# Autodesk Inventor assembly: 0329
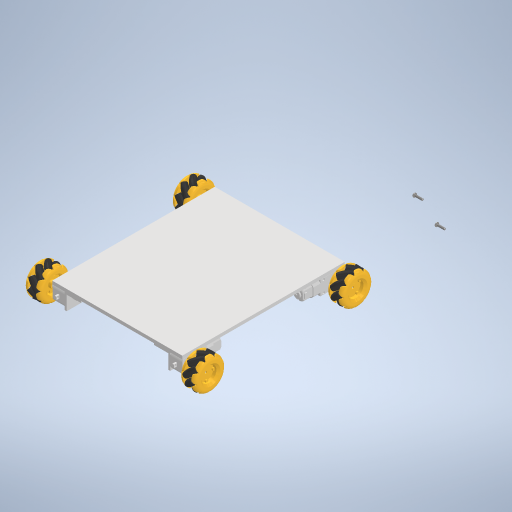
[picture p0: Inventor's stored thumbnail of the model, 512x512]
Saved by Autodesk Inventor 2023.2 (Build 272271030, 271C)
## iProperties
Created: 2023-03-29
Part Number: 0329
Document SubType Name: Assembly
Designer: kao91
Author: kao91
## Documents named in this file (9)
- C:\Users\kao91\Desktop\Mecharonic_practice\0329.iam
- C:\Users\kao91\Desktop\Mecharonic_practice\dc-motor-gearbox-tt-motor-1.snapshot.2\DC Motor Gearbox\DC Motor Gearbox.ipt
- C:\Users\kao91\Desktop\Mecharonic_practice\platform.ipt
- C:\Users\kao91\Desktop\Mecharonic_practice\connector.ipt
- C:\Users\kao91\OneDrive\文件\Inventor\Content Center Files\R2023\en-US\AS 1427(05)\AS 1427 - M3 x 12(5) II.ipt
- C:\Users\kao91\Desktop\Mecharonic_practice\df-robot-48mm-mecanum-wheel-left-side-1.snapshot.2\Mecanum Left v5\Mecanum Left v5.ipt
- C:\Users\kao91\Desktop\Mecharonic_practice\df-robot-48mm-mecanum-wheel-left-side-1.snapshot.2\Mecanum Left v5\Mecanum Ra.ipt
- C:\Users\kao91\Desktop\Mecharonic_practice\df-robot-48mm-mecanum-wheel-left-side-1.snapshot.2\Mecanum Left v5\Mecanum Rb.ipt
- C:\Users\kao91\Desktop\Mecharonic_practice\motor_to_mecanum_connector.ipt
## Components (19 placed, 8 different names)
1. platform:1 — Mate:1, Mate:2, Mate:3, Mate:4, Flush:2, Flush:3, Mate:5, Mate:7, Mate:9, Mate:11, Flush:4, Flush:5, Flush:6, Flush:7, Flush:8
2. connector:1 — Flush:3, Mate:5, Mate:6
3. connector:2 — Mate:7, Mate:8
4. connector:3 — Mate:9, Flush:5, Mate:13
5. connector:4 — Mate:11, Flush:4, Mate:14
6. AS 1427 H - Metric M3 x 12:1
7. AS 1427 H - Metric M3 x 12:2
8. DC Motor Gearbox:3 — Mate:3, Mate:13, Flush:8, Cylindrical:4, Mate:16, Flush:9
9. motor_to_mecanum_connector:4 — Cylindrical:4, Mate:16, Cylindrical:7, Mate:20
10. Mecanum Left v5:2 — Cylindrical:7, Mate:20
11. DC Motor Gearbox:1 — Mate:1, Mate:8, Flush:6, Cylindrical:2, Mate:18, Flush:10
12. motor_to_mecanum_connector:1 — Cylindrical:2, Mate:18, Cylindrical:8, Mate:22
13. Mecanum Left v5:1 — Cylindrical:8, Mate:22
14. DC Motor Gearbox:4 — Mate:4, Mate:14, Flush:7, Cylindrical:3, Mate:17, Flush:9
15. motor_to_mecanum_connector:3 — Cylindrical:3, Mate:17, Cylindrical:5, Mate:19
16. Mecanum Ra:1 — Cylindrical:5, Mate:19
17. DC Motor Gearbox:2 — Mate:2, Flush:2, Mate:6, Cylindrical:1, Mate:15, Flush:10
18. motor_to_mecanum_connector:2 — Cylindrical:1, Mate:15, Cylindrical:6, Mate:21
19. Mecanum Rb:1 — Cylindrical:6, Mate:21
## Relationships (37: Mate 20, Flush 9, CylindricalJoint 8)
- Mate:1: platform:1 ↔ DC Motor Gearbox:1
- Mate:2: platform:1 ↔ DC Motor Gearbox:2
- Mate:3: platform:1 ↔ DC Motor Gearbox:3
- Mate:4: platform:1 ↔ DC Motor Gearbox:4
- Flush:2: platform:1 ↔ DC Motor Gearbox:2
- Flush:3: platform:1 ↔ connector:1
- Mate:5: platform:1 ↔ connector:1
- Mate:6: connector:1 ↔ DC Motor Gearbox:2
- Mate:7: platform:1 ↔ connector:2
- Mate:8: connector:2 ↔ DC Motor Gearbox:1
- Mate:9: platform:1 ↔ connector:3
- Mate:11: platform:1 ↔ connector:4
- Flush:4: platform:1 ↔ connector:4
- Flush:5: platform:1 ↔ connector:3
- Flush:6: platform:1 ↔ DC Motor Gearbox:1
- Mate:13: connector:3 ↔ DC Motor Gearbox:3
- Mate:14: connector:4 ↔ DC Motor Gearbox:4
- Flush:7: platform:1 ↔ DC Motor Gearbox:4
- Cylindrical:1: DC Motor Gearbox:2 ↔ motor_to_mecanum_connector:2
- Mate:15: DC Motor Gearbox:2 ↔ motor_to_mecanum_connector:2
- Cylindrical:2: DC Motor Gearbox:1 ↔ motor_to_mecanum_connector:1
- Cylindrical:3: DC Motor Gearbox:4 ↔ motor_to_mecanum_connector:3
- Flush:8: platform:1 ↔ DC Motor Gearbox:3
- Cylindrical:4: DC Motor Gearbox:3 ↔ motor_to_mecanum_connector:4
- Mate:16: DC Motor Gearbox:3 ↔ motor_to_mecanum_connector:4
- Mate:17: DC Motor Gearbox:4 ↔ motor_to_mecanum_connector:3
- Mate:18: DC Motor Gearbox:1 ↔ motor_to_mecanum_connector:1
- Cylindrical:5: motor_to_mecanum_connector:3 ↔ Mecanum Ra:1
- Mate:19: motor_to_mecanum_connector:3 ↔ Mecanum Ra:1
- Cylindrical:6: motor_to_mecanum_connector:2 ↔ Mecanum Rb:1
- Cylindrical:7: motor_to_mecanum_connector:4 ↔ Mecanum Left v5:2
- Cylindrical:8: motor_to_mecanum_connector:1 ↔ Mecanum Left v5:1
- Mate:20: motor_to_mecanum_connector:4 ↔ Mecanum Left v5:2
- Mate:21: motor_to_mecanum_connector:2 ↔ Mecanum Rb:1
- Mate:22: motor_to_mecanum_connector:1 ↔ Mecanum Left v5:1
- Flush:9: DC Motor Gearbox:3 ↔ DC Motor Gearbox:4
- Flush:10: DC Motor Gearbox:1 ↔ DC Motor Gearbox:2
